# Autodesk Inventor assembly: A_Airbert
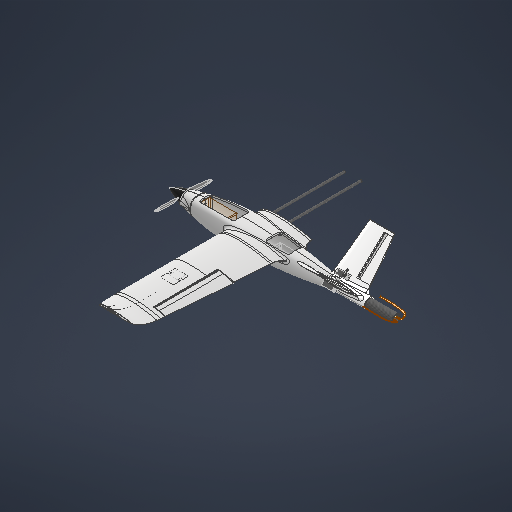
[picture p0: Inventor's stored thumbnail of the model, 512x512]
Saved by Autodesk Inventor 2026 (Build 300175000, 175)
## iProperties
Created: 2025-08-22
Part Number: A_Airbert
Document SubType Name: Assembly
Designer: FAL
Mass: 1703.33 g
Surface Area: 6443.47 cm^2
Volume: 1596.75 cm^3
Density: 1.06675 g/cm^3
Author: FAL
## Documents named in this file (35)
- C:\Users\FAL\Projekte\Git\AEROLAB\01_AIRCRAFTS\AIR-BERT\CAD\A_Airbert.iam
- C:\Users\FAL\Projekte\Git\AEROLAB\01_AIRCRAFTS\AIR-BERT\CAD\P_Fuselage.ipt
- C:\Users\FAL\Projekte\Git\AEROLAB\01_AIRCRAFTS\AIR-BERT\CAD\P_Carbon_Pipe_Back.ipt
- C:\Users\FAL\Projekte\Git\AEROLAB\01_AIRCRAFTS\AIR-BERT\CAD\extern\P_AP-PR-006_6-2_LH.ipt
- C:\Users\FAL\Projekte\Git\AEROLAB\01_AIRCRAFTS\AIR-BERT\CAD\P_aft_V.ipt
- C:\Users\FAL\Projekte\Git\AEROLAB\01_AIRCRAFTS\AIR-BERT\CAD\extern\P_Akku_Dummy.ipt
- C:\Users\FAL\Projekte\Git\AEROLAB\01_AIRCRAFTS\AIR-BERT\CAD\P_aft_T.ipt
- P_aft_T.ipt
- C:\Users\FAL\Projekte\Git\AEROLAB\01_AIRCRAFTS\AIR-BERT\CAD\extern\P_BLDC_2200KV.ipt
- C:\Users\FAL\Projekte\Git\AEROLAB\01_AIRCRAFTS\AIR-BERT\CAD\extern\P_Receiver_Radiolink.ipt
- C:\Users\FAL\Projekte\Git\AEROLAB\01_AIRCRAFTS\AIR-BERT\CAD\extern\P_ESC_40A.ipt
- C:\Users\FAL\Projekte\Git\AEROLAB\01_AIRCRAFTS\AIR-BERT\CAD\P_aft_X.ipt
- P_aft_X.ipt
- C:\Users\FAL\Projekte\Git\AEROLAB\01_AIRCRAFTS\AIR-BERT\CAD\P_MotorNose.ipt
- C:\Users\FAL\Projekte\Git\AEROLAB\01_AIRCRAFTS\AIR-BERT\CAD\P_Fuselage_cuts.ipt
- P_Fuselage_Cuts.ipt
- C:\Users\FAL\Projekte\Git\AEROLAB\01_AIRCRAFTS\AIR-BERT\CAD\P_Fuselage_Body.ipt
- C:\Users\FAL\Projekte\Git\AEROLAB\01_AIRCRAFTS\AIR-BERT\CAD\P_Fuselage_Nose.ipt
- C:\Users\FAL\Projekte\Git\AEROLAB\01_AIRCRAFTS\AIR-BERT\CAD\extern\P_Servo_SIMPROP.ipt
- C:\Users\FAL\Projekte\Git\AEROLAB\01_AIRCRAFTS\AIR-BERT\CAD\P_Wing_inner.ipt
- C:\Users\FAL\Projekte\Git\AEROLAB\01_AIRCRAFTS\AIR-BERT\CAD\P_Wing_mid.ipt
- C:\Users\FAL\Projekte\Git\AEROLAB\01_AIRCRAFTS\AIR-BERT\CAD\P_Wing_winglet.ipt
- C:\Users\FAL\Projekte\Git\AEROLAB\01_AIRCRAFTS\AIR-BERT\CAD\P_Wing_aileron.ipt
- C:\Users\FAL\Projekte\Git\AEROLAB\01_AIRCRAFTS\AIR-BERT\CAD\P_Fuselage_cap_front.ipt
- C:\Users\FAL\Projekte\Git\AEROLAB\01_AIRCRAFTS\AIR-BERT\CAD\P_Wing_Carbonpipe_A.ipt
- C:\Users\FAL\Projekte\Git\AEROLAB\01_AIRCRAFTS\AIR-BERT\CAD\P_Fuselage_cap_mid.ipt
- C:\Users\FAL\Projekte\Git\AEROLAB\01_AIRCRAFTS\AIR-BERT\CAD\P_Wing_mid_servocap.ipt
- C:\Users\FAL\Projekte\Git\AEROLAB\01_AIRCRAFTS\AIR-BERT\CAD\extern\P_Servo_SIMPROP_lever.ipt
- C:\Users\FAL\Projekte\Git\AEROLAB\01_AIRCRAFTS\AIR-BERT\CAD\P_Wing_mid_servolink.ipt
- C:\Users\FAL\Projekte\Git\AEROLAB\01_AIRCRAFTS\AIR-BERT\CAD\P_Wing_winglet_LEDcap.ipt
- C:\Users\FAL\Projekte\Git\AEROLAB\01_AIRCRAFTS\AIR-BERT\CAD\extern\P_Servo_SIMPROP_27x12.ipt
- C:\Users\FAL\Projekte\Git\AEROLAB\01_AIRCRAFTS\AIR-BERT\CAD\P_Harnes.ipt
- C:\Users\FAL\Projekte\Git\AEROLAB\01_AIRCRAFTS\AIR-BERT\CAD\P_aft_V_rudder.ipt
- C:\Users\FAL\Projekte\Git\AEROLAB\01_AIRCRAFTS\AIR-BERT\CAD\P_aft_V_rudder_MIR.ipt
- C:\Users\FAL\Projekte\Git\AEROLAB\01_AIRCRAFTS\AIR-BERT\CAD\P_Fuselage_Body_groundplate.ipt
## Components (35 placed, 31 different names)
1. P_Servo_SIMPROP_lever:1 — Passend:38, Passend:39, Passend:41, Tangential:1
2. P_Servo_SIMPROP:3 — Passend:36, Passend:37, Passend:38, Passend:39, Passend:40
3. P_AP-PR-006_6-2_LH:1 — Passend:14
4. P_MotorNose:1 — Passend:22
5. P_Akku_Dummy:1 — Passend:7
6. P_ESC_40A:1
7. P_Receiver_Radiolink:1
8. P_BLDC_2200KV:1 — Passend:12, Passend:31, Passend:32
9. P_Servo_SIMPROP_27x12:1 — Passend:49, Passend:53, Passend:55, Passend:59, Passend:60
10. P_Servo_SIMPROP_27x12:2 — Passend:50, Passend:54, Passend:56, Passend:57, Passend:58
11. P_Servo_SIMPROP_lever:4 — Passend:53, Passend:55
12. P_Servo_SIMPROP_lever:5 — Passend:54, Passend:56
13. P_aft_V_rudder_MIR:1 — Passend:64, Passend:65
14. P_aft_V_rudder:1 — Passend:61, Passend:62
15. P_Carbon_Pipe_Back:1 — Passend:6, Fluchtend:9, Passend:10, Fluchtend:10, Passend:15, Passend:16, Passend:21, Passend:28
16. P_aft_V:1 — Passend:6, Fluchtend:8, Fluchtend:9, Passend:49, Passend:50, Passend:57, Passend:58, Passend:59, Passend:60, Passend:61, Passend:62, Passend:64, Passend:65
17. P_aft_T:1 — Passend:9, Passend:10, Fluchtend:10
18. P_aft_X:1 — Passend:18, Passend:21, Passend:28
19. P_Fuselage_cap_front:1 — Fluchtend:53, Fluchtend:54, Fluchtend:55
20. P_Fuselage_cap_mid:1 — Fluchtend:58, Fluchtend:59, Fluchtend:60
21. P_Fuselage_Nose:1 — Fluchtend:32, Fluchtend:42, Fluchtend:43
22. P_Fuselage_Body:1 — Fluchtend:28, Fluchtend:29, Fluchtend:30, Passend:29, Passend:30, Passend:31
23. P_Fuselage:2 — Fluchtend:11, Fluchtend:12, Fluchtend:13, Passend:15, Passend:16
24. P_Fuselage_Cuts:1 — Fluchtend:14, Fluchtend:15, Fluchtend:16
25. P_Fuselage_Body_groundplate:1 — Fluchtend:73, Fluchtend:74, Fluchtend:75
26. P_Wing_mid_servocap:1 — Fluchtend:64, Fluchtend:65, Fluchtend:66
27. P_Wing_winglet:1 — Fluchtend:39, Fluchtend:40, Fluchtend:41
28. P_Wing_mid:1 — Fluchtend:36, Fluchtend:37, Fluchtend:38, Passend:36, Passend:37, Passend:40, Passend:42
29. P_Wing_aileron:1 — Fluchtend:44, Fluchtend:45, Fluchtend:46, Passend:42, Passend:63
30. P_Wing_mid_servolink:1 — Passend:41, Tangential:1
31. P_Wing_inner:1 — Fluchtend:33, Fluchtend:34, Fluchtend:35, Passend:63
32. P_Wing_Carbonpipe_A:1 — Passend:29, Fluchtend:56
33. P_Wing_Carbonpipe_A:2 — Fluchtend:57, Passend:30
34. P_Wing_winglet_LEDcap:1 — Fluchtend:67, Fluchtend:68, Fluchtend:69
35. P_Harnes:1 — Fluchtend:70, Fluchtend:71, Fluchtend:72
## Relationships (86: Flush 47, Mate 38, Tangent 1)
- Passend:6 [Mate]: P_Carbon_Pipe_Back:1 ↔ P_aft_V:1
- Fluchtend:8 [Flush]: P_aft_V:1
- Passend:7 [Mate]: P_Akku_Dummy:1
- Fluchtend:9 [Flush] (70 mm): P_Carbon_Pipe_Back:1 ↔ P_aft_V:1
- Passend:9 [Mate]: P_aft_T:1
- Passend:10 [Mate]: P_Carbon_Pipe_Back:1 ↔ P_aft_T:1
- Fluchtend:10 [Flush]: P_Carbon_Pipe_Back:1 ↔ P_aft_T:1
- Passend:12 [Mate]: P_BLDC_2200KV:1
- Passend:14 [Mate]: P_AP-PR-006_6-2_LH:1
- Fluchtend:11 [Flush]: P_Fuselage:2
- Fluchtend:12 [Flush]: P_Fuselage:2
- Fluchtend:13 [Flush]: P_Fuselage:2
- Passend:15 [Mate]: P_Carbon_Pipe_Back:1 ↔ P_Fuselage:2
- Passend:16 [Mate] (-60 mm): P_Carbon_Pipe_Back:1 ↔ P_Fuselage:2
- Passend:18 [Mate]: P_aft_X:1
- Passend:21 [Mate]: P_Carbon_Pipe_Back:1 ↔ P_aft_X:1
- Passend:22 [Mate]: P_MotorNose:1
- Fluchtend:14 [Flush]: P_Fuselage_Cuts:1
- Fluchtend:15 [Flush]: P_Fuselage_Cuts:1
- Fluchtend:16 [Flush]: P_Fuselage_Cuts:1
- Fluchtend:28 [Flush]: P_Fuselage_Body:1
- Fluchtend:29 [Flush]: P_Fuselage_Body:1
- Fluchtend:30 [Flush]: P_Fuselage_Body:1
- Fluchtend:32 [Flush]: P_Fuselage_Nose:1
- Fluchtend:42 [Flush]: P_Fuselage_Nose:1
- Fluchtend:43 [Flush]: P_Fuselage_Nose:1
- Passend:28 [Mate]: P_Carbon_Pipe_Back:1 ↔ P_aft_X:1
- Fluchtend:33 [Flush]: P_Wing_inner:1
- Fluchtend:34 [Flush]: P_Wing_inner:1
- Fluchtend:35 [Flush]: P_Wing_inner:1
- Fluchtend:36 [Flush]: P_Wing_mid:1
- Fluchtend:37 [Flush]: P_Wing_mid:1
- Fluchtend:38 [Flush]: P_Wing_mid:1
- Fluchtend:39 [Flush]: P_Wing_winglet:1
- Fluchtend:40 [Flush]: P_Wing_winglet:1
- Fluchtend:41 [Flush]: P_Wing_winglet:1
- Fluchtend:44 [Flush]: P_Wing_aileron:1
- Fluchtend:45 [Flush]: P_Wing_aileron:1
- Fluchtend:46 [Flush]: P_Wing_aileron:1
- Fluchtend:53 [Flush]: P_Fuselage_cap_front:1
- Fluchtend:54 [Flush]: P_Fuselage_cap_front:1
- Fluchtend:55 [Flush]: P_Fuselage_cap_front:1
- Passend:29 [Mate]: P_Fuselage_Body:1 ↔ P_Wing_Carbonpipe_A:1
- Fluchtend:56 [Flush]: P_Wing_Carbonpipe_A:1
- Fluchtend:57 [Flush]: P_Wing_Carbonpipe_A:2
- Passend:30 [Mate]: P_Fuselage_Body:1 ↔ P_Wing_Carbonpipe_A:2
- Passend:31 [Mate]: P_BLDC_2200KV:1 ↔ P_Fuselage_Body:1
- Passend:32 [Mate]: P_BLDC_2200KV:1
- Fluchtend:58 [Flush]: P_Fuselage_cap_mid:1
- Fluchtend:59 [Flush]: P_Fuselage_cap_mid:1
- Fluchtend:60 [Flush]: P_Fuselage_cap_mid:1
- Passend:36 [Mate]: P_Servo_SIMPROP:3 ↔ P_Wing_mid:1
- Passend:37 [Mate]: P_Servo_SIMPROP:3 ↔ P_Wing_mid:1
- Fluchtend:64 [Flush]: P_Wing_mid_servocap:1
- Fluchtend:65 [Flush]: P_Wing_mid_servocap:1
- Fluchtend:66 [Flush]: P_Wing_mid_servocap:1
- Passend:38 [Mate]: P_Servo_SIMPROP_lever:1 ↔ P_Servo_SIMPROP:3
- Passend:39 [Mate]: P_Servo_SIMPROP_lever:1 ↔ P_Servo_SIMPROP:3
- Passend:40 [Mate]: P_Servo_SIMPROP:3 ↔ P_Wing_mid:1
- Passend:41 [Mate]: P_Servo_SIMPROP_lever:1 ↔ P_Wing_mid_servolink:1
- Tangential:1: P_Servo_SIMPROP_lever:1 ↔ P_Wing_mid_servolink:1
- Passend:42 [Mate]: P_Wing_mid:1 ↔ P_Wing_aileron:1
- Fluchtend:67 [Flush]: P_Wing_winglet_LEDcap:1
- Fluchtend:68 [Flush]: P_Wing_winglet_LEDcap:1
- Fluchtend:69 [Flush]: P_Wing_winglet_LEDcap:1
- Passend:49 [Mate]: P_Servo_SIMPROP_27x12:1 ↔ P_aft_V:1
- Passend:50 [Mate]: P_Servo_SIMPROP_27x12:2 ↔ P_aft_V:1
- Passend:53 [Mate]: P_Servo_SIMPROP_27x12:1 ↔ P_Servo_SIMPROP_lever:4
- Passend:54 [Mate]: P_Servo_SIMPROP_27x12:2 ↔ P_Servo_SIMPROP_lever:5
- Passend:55 [Mate]: P_Servo_SIMPROP_27x12:1 ↔ P_Servo_SIMPROP_lever:4
- Passend:56 [Mate]: P_Servo_SIMPROP_27x12:2 ↔ P_Servo_SIMPROP_lever:5
- Passend:57 [Mate]: P_Servo_SIMPROP_27x12:2 ↔ P_aft_V:1
- Passend:58 [Mate]: P_Servo_SIMPROP_27x12:2 ↔ P_aft_V:1
- Passend:59 [Mate]: P_Servo_SIMPROP_27x12:1 ↔ P_aft_V:1
- Passend:60 [Mate]: P_Servo_SIMPROP_27x12:1 ↔ P_aft_V:1
- Fluchtend:70 [Flush]: P_Harnes:1
- Fluchtend:71 [Flush]: P_Harnes:1
- Fluchtend:72 [Flush]: P_Harnes:1
- Passend:61 [Mate]: P_aft_V_rudder:1 ↔ P_aft_V:1
- Passend:62 [Mate]: P_aft_V_rudder:1 ↔ P_aft_V:1
- Passend:63 [Mate] (1 mm): P_Wing_aileron:1 ↔ P_Wing_inner:1
- Fluchtend:73 [Flush]: P_Fuselage_Body_groundplate:1
- Fluchtend:74 [Flush]: P_Fuselage_Body_groundplate:1
- Fluchtend:75 [Flush]: P_Fuselage_Body_groundplate:1
- Passend:64 [Mate]: P_aft_V_rudder_MIR:1 ↔ P_aft_V:1
- Passend:65 [Mate]: P_aft_V_rudder_MIR:1 ↔ P_aft_V:1
